# Autodesk Inventor assembly: ASY GBK 3120 central wall shield 2
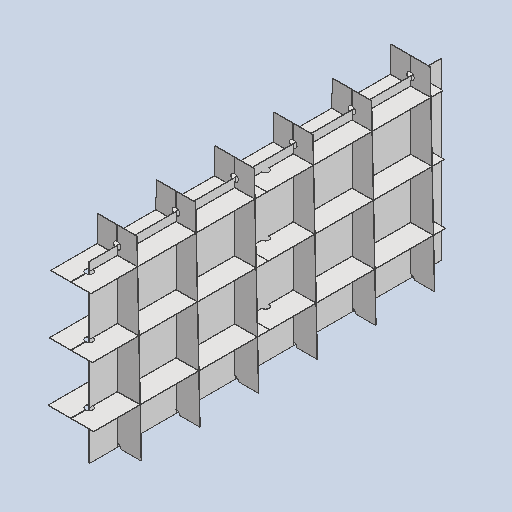
[picture p0: Inventor's stored thumbnail of the model, 512x512]
Saved by Autodesk Inventor 2026.3 (Build 303398000, 398)
## iProperties
Created: 2026-05-19
Part Number: ASY GBK 3120 central wall shield 2
Document SubType Name: Assembly
Designer: pokla
Mass: 174041 g
Surface Area: 113034 cm^2
Volume: 22170.8 cm^3
Density: 7.85 g/cm^3
Stock Number: 3120
Author: admin
## Documents named in this file (8)
- C:\Users\admin\Documents\Inventor\GBK-Gubkinskiy\ASY GBK 3120 central wall shield 2.iam
- C:\Users\admin\Documents\Inventor\GBK-Gubkinskiy\GBK 0101 main rib.ipt
- C:\Users\admin\Documents\Inventor\GBK-Gubkinskiy\GBK 3122 shield 2.ipt
- C:\Users\admin\Documents\Inventor\GBK-Gubkinskiy\GBK 3112 central main rib_CPY.ipt
- GBK 3112 central main rib_CPY.ipt
- C:\Users\admin\Documents\Inventor\GBK-Gubkinskiy\GBK 3113 stringer 1.ipt
- C:\Users\admin\Documents\Inventor\GBK-Gubkinskiy\GBK 3114 stringer 2.ipt
- C:\Users\admin\Documents\Inventor\GBK-Gubkinskiy\GBK 3115 stringer 3.ipt
## Components (25 placed, 5 different names)
1. GBK 3113 stringer 1:1 — Rigid:1, Rigid:10
2. GBK 3122 shield 2:1 — Mate:1, Flush:1, Mate:2, Flush:3, Mate:5, Flush:2, Mate:4, Flush:6
3. GBK 3114 stringer 2:1 — Rigid:2, Rigid:11
4. GBK 3115 stringer 3:1 — Rigid:3, Rigid:12
5. GBK 3113 stringer 1:2 — Rigid:6, Rigid:7
6. GBK 3114 stringer 2:2 — Rigid:5, Rigid:8
7. GBK 3115 stringer 3:2 — Rigid:6, Rigid:9, Flush:6
8. GBK 3113 stringer 1:3 — Rigid:7
9. GBK 3114 stringer 2:3 — Rigid:8
10. GBK 3115 stringer 3:3 — Rigid:9
11. GBK 3113 stringer 1:4 — Rigid:10
12. GBK 3114 stringer 2:4 — Rigid:11
13. GBK 3115 stringer 3:4 — Rigid:12
14. GBK 3112 central main rib_CPY:1 — Flush:2, Mate:4, Flush:4, Rigid:6, Rigid:5, Rigid:6
15. GBK 3112 central main rib_CPY:2 — Flush:3, Mate:5, Flush:4, Rigid:3, Rigid:2, Rigid:1
16. GBK 3112 central main rib_CPY:3
17. GBK 3112 central main rib_CPY:4
18. GBK 3112 central main rib_CPY:5
19. GBK 3112 central main rib_CPY:6
20. GBK 3112 central main rib_CPY:7
21. GBK 3112 central main rib_CPY:8
22. GBK 3112 central main rib_CPY:9
23. GBK 3112 central main rib_CPY:10
24. GBK 3112 central main rib_CPY:11
25. GBK 3112 central main rib_CPY:12
## Component patterns: (6 elements, first: GBK 3112 central main rib_CPY:1 + GBK 3112 central main rib_CPY:2)
## Relationships (21: WeldJoint 12, Flush 5, Mate 4)
- Mate:1: GBK 3122 shield 2:1
- Flush:1: GBK 3122 shield 2:1
- Mate:2: GBK 3122 shield 2:1
- Flush:3: GBK 3122 shield 2:1 ↔ GBK 3112 central main rib_CPY:2
- Mate:5: GBK 3122 shield 2:1 ↔ GBK 3112 central main rib_CPY:2
- Flush:2: GBK 3122 shield 2:1 ↔ GBK 3112 central main rib_CPY:1
- Mate:4: GBK 3122 shield 2:1 ↔ GBK 3112 central main rib_CPY:1
- Flush:4: GBK 3112 central main rib_CPY:1 ↔ GBK 3112 central main rib_CPY:2
- Rigid:3 [WeldJoint] (4 mm): GBK 3115 stringer 3:1 ↔ GBK 3112 central main rib_CPY:2
- Rigid:2 [WeldJoint] (4 mm): GBK 3114 stringer 2:1 ↔ GBK 3112 central main rib_CPY:2
- Rigid:1 [WeldJoint] (4 mm): GBK 3113 stringer 1:1 ↔ GBK 3112 central main rib_CPY:2
- Rigid:6 [WeldJoint] (4 mm): GBK 3113 stringer 1:2 ↔ GBK 3112 central main rib_CPY:1
- Rigid:5 [WeldJoint] (4 mm): GBK 3114 stringer 2:2 ↔ GBK 3112 central main rib_CPY:1
- Rigid:6 [WeldJoint] (4 mm): GBK 3115 stringer 3:2 ↔ GBK 3112 central main rib_CPY:1
- Rigid:7 [WeldJoint] (1 mm): GBK 3113 stringer 1:2 ↔ GBK 3113 stringer 1:3
- Rigid:8 [WeldJoint] (1 mm): GBK 3114 stringer 2:2 ↔ GBK 3114 stringer 2:3
- Rigid:9 [WeldJoint] (1 mm): GBK 3115 stringer 3:2 ↔ GBK 3115 stringer 3:3
- Rigid:10 [WeldJoint] (1 mm): GBK 3113 stringer 1:1 ↔ GBK 3113 stringer 1:4
- Rigid:11 [WeldJoint] (1 mm): GBK 3114 stringer 2:1 ↔ GBK 3114 stringer 2:4
- Rigid:12 [WeldJoint] (1 mm): GBK 3115 stringer 3:1 ↔ GBK 3115 stringer 3:4
- Flush:6 (155 mm): GBK 3122 shield 2:1 ↔ GBK 3115 stringer 3:2
## Named parameters: основание_длина_нижнего = 200 mm, основание_длина_верхнего = 100 mm, стрингер_глубина_1 = 190.70056 mm, стрингер_глубина_2 = 179.35977 mm, стрингер_глубина_3 = 168.01899 mm, стрингер_глубина_4 = 156.6782 mm, стрингер_глубина_5 = 145.33742 mm, стрингер_глубина_6 = 133.99663 mm, стрингер_глубина_7 = 122.65585 mm, стрингер_глубина_8 = 111.31507 mm, Лист_ширина = 1480 mm, ребро_усилителей = 60 mm, паз_под_стрингер_глубина = 70 mm, паз_под_стрингер_толщина = 5 mm, отступ_от_пола_до_первого_стрингера = 410 mm, шаг_стрингеров = 500 mm, радиус_выреза_под_сварку = 30 mm, нахлест_шпангоутов_1_2 = 150 mm, нахлест_шпангоутов_2_3 = 120 mm, Стрингер_длина = 1489.5 mm, Лист_длина = 2980 mm, Шаг_шпангоутов = 496.66667 mm
